# Autodesk Inventor assembly: Detection Aseembly with Stages
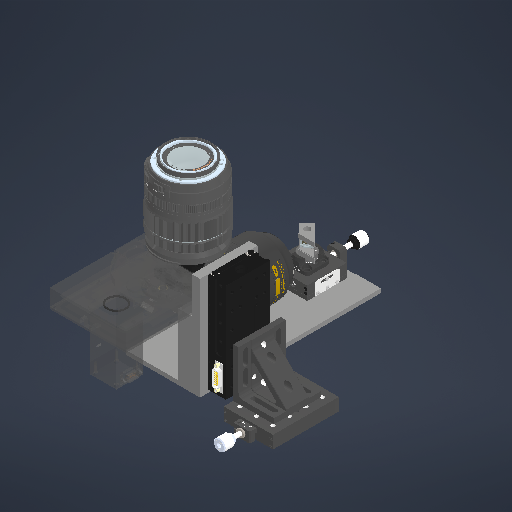
[picture p0: Inventor's stored thumbnail of the model, 512x512]
Saved by Autodesk Inventor 2026 (Build 300175000, 175)
## iProperties
Created: 2026-03-04
Part Number: Detection Aseembly with Stages
Document SubType Name: Assembly
Designer: FiolkaLab
Author: FiolkaLab
## Documents named in this file (4)
- E:\Muaaz\Baseplate\ASLM_DvOPM System Assembly\Detection Aseembly with Stages.iam
- E:\Muaaz\Baseplate\ASLM_DvOPM System Assembly\PT1B-Step\PT1B-Step\PT1B-Step.ipt
- E:\Muaaz\Baseplate\ASLM_DvOPM System Assembly\AP90-Step\AP90-Step\AP90-Step.ipt
- E:\Muaaz\Baseplate\Detection\V2 Baseplate Detection Aseembly.iam
## Components (4 placed, 3 different names)
1. PT1B-Step:1 — Angle:1, Mate:1, Mate:2
2. PT1B-Step:2 — Angle:1, Mate:1, Mate:2, Mate:3, Flush:1
3. AP90-Step:1 — Mate:3, Mate:4, Mate:5, Flush:1
4. V2 Baseplate Detection Aseembly:1 [sub-assembly] — Mate:4, Mate:5
## Relationships (7: Mate 5, Angle 1, Flush 1)
- Angle:1 (180 deg): PT1B-Step:1 ↔ PT1B-Step:2
- Mate:1: PT1B-Step:1 ↔ PT1B-Step:2
- Mate:2: PT1B-Step:1 ↔ PT1B-Step:2
- Mate:3: PT1B-Step:2 ↔ AP90-Step:1
- Mate:4: AP90-Step:1 ↔ V2 Baseplate Detection Aseembly:1
- Mate:5: AP90-Step:1 ↔ V2 Baseplate Detection Aseembly:1
- Flush:1: PT1B-Step:2 ↔ AP90-Step:1
